# Autodesk Inventor assembly: DHT_sestava
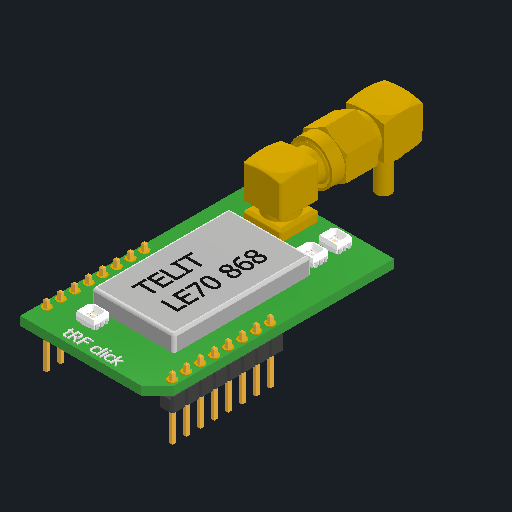
[picture p0: Inventor's stored thumbnail of the model, 512x512]
Saved by Autodesk Inventor 2022 (Build 260153000, 153)
## iProperties
Created: 2022-03-19
Part Number: DHT_sestava
Document SubType Name: Assembly
Designer: dvorakj
Author: dvorakj
## Documents named in this file (7)
- C:\Users\dvorakj\Documents\Inventor\Bakalarka\Clicks\tRF\tRF sestava.iam
- C:\Users\dvorakj\Documents\Inventor\Bakalarka\Clicks\Pin Header\61300811121 (rev1).iam
- C:\Users\dvorakj\Documents\Inventor\Bakalarka\Clicks\tRF\tRF pcb.ipt
- C:\Users\dvorakj\Documents\Inventor\Bakalarka\Clicks\tRF\SMA\SMA ANGLED.ipt
- C:\Users\dvorakj\Documents\Inventor\Bakalarka\Clicks\DHT22\Telit.ipt
- C:\Users\dvorakj\Documents\Inventor\Bakalarka\Clicks\tRF\LED\Download_Step_150352M173300 (rev1).iam
- C:\Users\dvorakj\Documents\Inventor\Bakalarka\SMA_RA\User Library-SMA_JACK.ipt
## Components (9 placed, 6 different names)
1. 61300811121 (rev1):1 [sub-assembly] — Mate:3
2. 61300811121 (rev1):2 [sub-assembly] — Mate:1, Mate:2
3. tRF pcb:1 — Mate:1, Mate:2, Mate:3, Mate:4, Flush:1, Flush:2, Flush:3, Mate:5, Mate:6, Mate:7
4. SMA ANGLED:1 — Mate:4, Flush:1, Flush:2, Mate:10, Mate:11, Mate:12
5. Telit:1 — Flush:3, Mate:8
6. Download_Step_150352M173300 (rev1):1 [sub-assembly] — Mate:5, Flush:4, Mate:9
7. Download_Step_150352M173300 (rev1):2 [sub-assembly] — Mate:6, Flush:4, Mate:8, Mate:9, Mate:10
8. Download_Step_150352M173300 (rev1):3 [sub-assembly] — Mate:7
9. User Library-SMA_JACK:1 — Mate:11, Mate:12
## Relationships (16: Mate 12, Flush 4)
- Mate:1: 61300811121 (rev1):2 ↔ tRF pcb:1
- Mate:2: 61300811121 (rev1):2 ↔ tRF pcb:1
- Mate:3: 61300811121 (rev1):1 ↔ tRF pcb:1
- Mate:4: tRF pcb:1 ↔ SMA ANGLED:1
- Flush:1 (5.4 mm): tRF pcb:1 ↔ SMA ANGLED:1
- Flush:2 (1 mm): tRF pcb:1 ↔ SMA ANGLED:1
- Flush:3: tRF pcb:1 ↔ Telit:1
- Mate:5: tRF pcb:1 ↔ Download_Step_150352M173300 (rev1):1
- Mate:6: tRF pcb:1 ↔ Download_Step_150352M173300 (rev1):2
- Mate:7: tRF pcb:1 ↔ Download_Step_150352M173300 (rev1):3
- Flush:4: Download_Step_150352M173300 (rev1):1 ↔ Download_Step_150352M173300 (rev1):2
- Mate:8 (1 mm): Telit:1 ↔ Download_Step_150352M173300 (rev1):2
- Mate:9 (1.5 mm): Download_Step_150352M173300 (rev1):1 ↔ Download_Step_150352M173300 (rev1):2
- Mate:10 (3.5 mm): SMA ANGLED:1 ↔ Download_Step_150352M173300 (rev1):2
- Mate:11: SMA ANGLED:1 ↔ User Library-SMA_JACK:1
- Mate:12 (-2 mm): SMA ANGLED:1 ↔ User Library-SMA_JACK:1
